# Autodesk Inventor assembly: Table
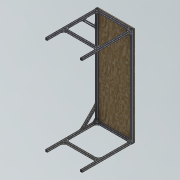
[picture p0: Inventor's stored thumbnail of the model, 180x180]
Saved by Autodesk Inventor 2020.2 (Build 242310000, 310)
## iProperties
Created: 2020-07-25
Part Number: Table
Document SubType Name: Assembly
Designer: JK
Author: JK
## Documents named in this file (6)
- C:\Users\JK\Documents\Inventor\Mesa\Table.iam
- C:\Users\JK\Documents\Inventor\Mesa\Topassembly.iam
- C:\Users\JK\Documents\Inventor\Mesa\Sideassembly.iam
- C:\Users\JK\Documents\Inventor\Mesa\diagonalstretcher.iam
- C:\Users\JK\Documents\Inventor\Mesa\Sideassembly_MIR.iam
- C:\Users\JK\Documents\Inventor\Mesa\diagonalstretcher_MIR.iam
## Components (5 placed, 5 different names)
1. Topassembly:1 [sub-assembly] — Flush:1, Flush:2, Mate:1, Mate:3, Mate:6, Flush:5, Flush:6, Mate:7
2. Sideassembly:1 [sub-assembly] — Flush:1, Flush:2, Mate:1, Mate:2, Flush:3, Mate:5
3. diagonalstretcher:1 [sub-assembly] — Mate:2, Flush:3, Mate:3
4. Sideassembly_MIR:1 [sub-assembly] — Flush:4, Mate:4, Mate:6, Flush:5, Flush:6
5. diagonalstretcher_MIR:1 [sub-assembly] — Flush:4, Mate:4, Mate:7
## Relationships (13: Mate 7, Flush 6)
- Flush:1: Topassembly:1 ↔ Sideassembly:1
- Flush:2: Topassembly:1 ↔ Sideassembly:1
- Mate:1: Topassembly:1 ↔ Sideassembly:1
- Mate:2: Sideassembly:1 ↔ diagonalstretcher:1
- Flush:3: Sideassembly:1 ↔ diagonalstretcher:1
- Mate:3: Topassembly:1 ↔ diagonalstretcher:1
- Flush:4: Sideassembly_MIR:1 ↔ diagonalstretcher_MIR:1
- Mate:4: Sideassembly_MIR:1 ↔ diagonalstretcher_MIR:1
- Mate:5: Sideassembly:1
- Mate:6: Topassembly:1 ↔ Sideassembly_MIR:1
- Flush:5: Topassembly:1 ↔ Sideassembly_MIR:1
- Flush:6: Topassembly:1 ↔ Sideassembly_MIR:1
- Mate:7: Topassembly:1 ↔ diagonalstretcher_MIR:1
